# Autodesk Inventor assembly: SE SiPM 8CH Org
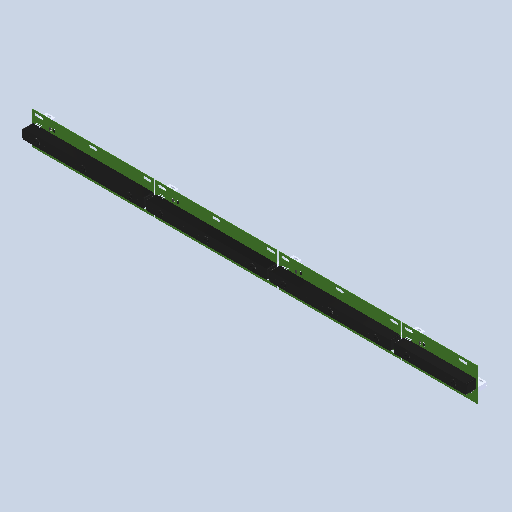
[picture p0: Inventor's stored thumbnail of the model, 512x512]
Saved by Autodesk Inventor 2024.2 (Build 282272000, 272)
## iProperties
Created: 2024-09-02
Part Number: SE SiPM 8CH Org
Document SubType Name: Assembly
Designer: ja.restrepo1
Author: ja.restrepo1
## Documents named in this file (5)
- I:\MICROMECANICA\ALTAS ENERGIAS\Deteccion de Muones\Detectores centelladores\Partes Detector Centellador\SE Tarjetas IC DC\SSE SiPM 8CH Org.iam
- I:\MICROMECANICA\ALTAS ENERGIAS\Deteccion de Muones\Detectores centelladores\Partes Detector Centellador\SE Tarjetas IC DC\SiPM 8Ch vf2_pcb\SiPM 8Ch vf2_pcb.iam
- I:\MICROMECANICA\ALTAS ENERGIAS\Deteccion de Muones\Detectores centelladores\Partes Detector Centellador\SE Tarjetas IC DC\PCB SiPM DC\SiPM 4CH 2X3 PCB.iam
- I:\MICROMECANICA\ALTAS ENERGIAS\Deteccion de Muones\Detectores centelladores\Partes Detector Centellador\SE Tarjetas IC DC\Guias SiPM\Guia fibra  SiPM 4Ch DC.ipt
- I:\MICROMECANICA\ALTAS ENERGIAS\Deteccion de Muones\Detectores centelladores\Partes Detector Centellador\SE Tarjetas IC DC\Guias SiPM\Guia fibra  SiPM 8Ch DC.ipt
## Components (8 placed, 4 different names)
1. SiPM 8Ch vf2_pcb:1 [sub-assembly] — Flush:1, Flush:4, Flush:5, Mate:2, Flush:6, Flush:7, Mate:4, Mate:8, Mate:9, Mate:10
2. SiPM 8Ch vf2_pcb:2 [sub-assembly] — Flush:1, Flush:2, Flush:3, Flush:4, Mate:1, Flush:5, Mate:2, Mate:3, Angle:1, Mate:11, Mate:12, Mate:13
3. SiPM 8Ch vf2_pcb:3 [sub-assembly] — Flush:2, Flush:3, Mate:3, Mate:14, Mate:15, Mate:16
4. SiPM 4CH 2X3 PCB:1 [sub-assembly] — Flush:6, Flush:7, Mate:4, Mate:5, Mate:6, Mate:7
5. Guia fibra  SiPM 4Ch DC:1 — Mate:5, Mate:6, Mate:7
6. Guia fibra  SiPM 8Ch DC:1 — Mate:8, Mate:9, Mate:10
7. Guia fibra  SiPM 8Ch DC:2 — Mate:11, Mate:12, Mate:13
8. Guia fibra  SiPM 8Ch DC:3 — Mate:14, Mate:15, Mate:16
## Relationships (24: Mate 16, Flush 7, Angle 1)
- Flush:1: SiPM 8Ch vf2_pcb:1 ↔ SiPM 8Ch vf2_pcb:2
- Flush:2: SiPM 8Ch vf2_pcb:2 ↔ SiPM 8Ch vf2_pcb:3
- Flush:3: SiPM 8Ch vf2_pcb:2 ↔ SiPM 8Ch vf2_pcb:3
- Flush:4: SiPM 8Ch vf2_pcb:1 ↔ SiPM 8Ch vf2_pcb:2
- Mate:1: SiPM 8Ch vf2_pcb:2
- Flush:5: SiPM 8Ch vf2_pcb:1 ↔ SiPM 8Ch vf2_pcb:2
- Mate:2 (2 mm): SiPM 8Ch vf2_pcb:1 ↔ SiPM 8Ch vf2_pcb:2
- Mate:3 (2 mm): SiPM 8Ch vf2_pcb:2 ↔ SiPM 8Ch vf2_pcb:3
- Angle:1 (0 deg): SiPM 8Ch vf2_pcb:2
- Flush:6: SiPM 8Ch vf2_pcb:1 ↔ SiPM 4CH 2X3 PCB:1
- Flush:7: SiPM 8Ch vf2_pcb:1 ↔ SiPM 4CH 2X3 PCB:1
- Mate:4 (2 mm): SiPM 8Ch vf2_pcb:1 ↔ SiPM 4CH 2X3 PCB:1
- Mate:5: SiPM 4CH 2X3 PCB:1 ↔ Guia fibra  SiPM 4Ch DC:1
- Mate:6: SiPM 4CH 2X3 PCB:1 ↔ Guia fibra  SiPM 4Ch DC:1
- Mate:7: SiPM 4CH 2X3 PCB:1 ↔ Guia fibra  SiPM 4Ch DC:1
- Mate:8: SiPM 8Ch vf2_pcb:1 ↔ Guia fibra  SiPM 8Ch DC:1
- Mate:9: SiPM 8Ch vf2_pcb:1 ↔ Guia fibra  SiPM 8Ch DC:1
- Mate:10: SiPM 8Ch vf2_pcb:1 ↔ Guia fibra  SiPM 8Ch DC:1
- Mate:11: SiPM 8Ch vf2_pcb:2 ↔ Guia fibra  SiPM 8Ch DC:2
- Mate:12: SiPM 8Ch vf2_pcb:2 ↔ Guia fibra  SiPM 8Ch DC:2
- Mate:13: SiPM 8Ch vf2_pcb:2 ↔ Guia fibra  SiPM 8Ch DC:2
- Mate:14: SiPM 8Ch vf2_pcb:3 ↔ Guia fibra  SiPM 8Ch DC:3
- Mate:15: SiPM 8Ch vf2_pcb:3 ↔ Guia fibra  SiPM 8Ch DC:3
- Mate:16: SiPM 8Ch vf2_pcb:3 ↔ Guia fibra  SiPM 8Ch DC:3
